# Autodesk Inventor assembly: Frame Assembly - Bade v1
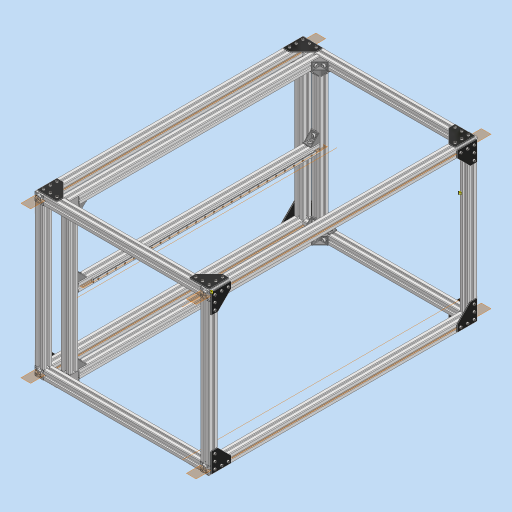
[picture p0: Inventor's stored thumbnail of the model, 512x512]
Saved by Autodesk Inventor 2023.2 (Build 272271000, 271)
## iProperties
Created: 2023-11-22
Part Number: Frame Assembly - Bade v1
Document SubType Name: Assembly
Designer: Nils Bade
Author: Nils Bade
## Documents named in this file (14)
- C:\Users\nilsb\Documents\Inventor\Projektarbeit-Bade\RatRig_Bade\Frame Assembly - Bade v1.iam
- C:\Users\nilsb\Documents\Inventor\Projektarbeit-Bade\RatRig_modified\T-SLOT 4040 B-Type 705mm.ipt
- C:\Users\nilsb\Documents\Inventor\Projektarbeit-Bade\RatRig_modified\T-SLOT 4040 B-Type 640mm.ipt
- C:\Users\nilsb\Documents\Inventor\Projektarbeit-Bade\RatRig_modified\T-SLOT 4040 B-Type 1207mm.ipt
- C:\Users\nilsb\Documents\Inventor\Projektarbeit-Bade\RatRig_modified\T-SLOT 4040 B-Type 1127mm.ipt
- C:\Users\nilsb\Documents\Inventor\Projektarbeit-Bade\RatRig_modified\Joining Plate for 4040 Assembly - A.iam
- C:\Users\nilsb\Documents\Inventor\Projektarbeit-Bade\RatRig_modified\Joining Plate for 4040 Assembly - B.iam
- C:\Users\nilsb\Documents\Inventor\Projektarbeit-Bade\RatRig_modified\Joining Plate for 4040 Assembly - C.iam
- C:\Users\nilsb\Documents\Inventor\Projektarbeit-Bade\RatRig_modified\Joining Plate for 4040 Assembly - A_mir.iam
- C:\Users\nilsb\Documents\Inventor\Projektarbeit-Bade\RatRig_modified\Joining Plate for 4040 Assembly - B_mir.iam
- C:\Users\nilsb\Documents\Inventor\Projektarbeit-Bade\RatRig_modified\Bracket - Cast 90 deg corner 4040 - Assembly.iam
- C:\Users\nilsb\Documents\Inventor\Projektarbeit-Bade\RatRig_modified\T-SLOT 4040 B-Type 1087mm.ipt
- C:\Users\nilsb\Documents\Inventor\Projektarbeit-Bade\RatRig_modified\MGN15 Linear Rail 1000mm - 4040 Assembly.iam
- C:\Users\nilsb\Documents\Inventor\Projektarbeit-Bade\RatRig_modified\MGN15 Linear Rail 550mm - 4040 Assembly.iam
## Components (54 placed, 13 different names)
1. T-SLOT 4040 B-Type 705mm:1 — Passend:1, Passend:2, Passend:3, Passend:6, Passend:7, Passend:8, Fluchtend:6, Fluchtend:8, Fluchtend:9, Fluchtend:14, Passend:14, Fluchtend:19, Fluchtend:20, Passend:15, Passend:20, Fluchtend:29, Passend:51, Passend:53, Passend:54, Passend:62, Passend:63, Passend:115, Passend:117, Passend:119, Fluchtend:39
2. T-SLOT 4040 B-Type 640mm:1 — Passend:6, Fluchtend:8, Passend:17, Fluchtend:22, Fluchtend:23, Passend:40, Passend:41, Passend:55, Passend:56, Passend:57
3. T-SLOT 4040 B-Type 640mm:2 — Passend:7, Fluchtend:9, Passend:9, Fluchtend:26, Fluchtend:27, Passend:108, Passend:110, Passend:111, Passend:113, Passend:114, Passend:116, Passend:123, Passend:125, Passend:139, Passend:140, Passend:141, Passend:142, Fluchtend:40
4. T-SLOT 4040 B-Type 640mm:3 — Passend:8, Fluchtend:6, Passend:9, Fluchtend:16, Passend:16, Fluchtend:21, Fluchtend:24, Passend:31, Passend:32, Passend:48, Passend:52
5. T-SLOT 4040 B-Type 705mm:2 — Fluchtend:14, Passend:18, Passend:19, Fluchtend:25, Passend:21, Fluchtend:28, Passend:49, Passend:50, Passend:58, Passend:59, Passend:70, Passend:71, Passend:74, Passend:75, Passend:120, Passend:122, Passend:124
6. T-SLOT 4040 B-Type 1207mm:1 — Passend:10, Fluchtend:20, Passend:15, Fluchtend:24, Passend:25, Fluchtend:36, Passend:28, Passend:29, Passend:30, Passend:46, Passend:60, Passend:61, Passend:67, Passend:82, Passend:84, Passend:85, Passend:86, Fluchtend:42, Fluchtend:46, Fluchtend:47, Passend:163, Passend:164
7. T-SLOT 4040 B-Type 1207mm:2 — Passend:12, Passend:17, Fluchtend:22, Passend:23, Fluchtend:32, Fluchtend:33, Passend:38, Passend:39, Passend:43, Passend:44, Passend:72, Passend:73, Passend:94, Passend:95, Passend:97, Passend:98
8. T-SLOT 4040 B-Type 1207mm:3 — Passend:13, Passend:16, Fluchtend:21, Passend:19, Fluchtend:25, Fluchtend:34, Passend:33, Passend:34, Passend:35, Passend:47, Passend:68, Passend:69, Passend:89, Passend:90, Passend:91, Passend:92, Fluchtend:43, Fluchtend:44, Fluchtend:48, Passend:162, Passend:165
9. T-SLOT 4040 B-Type 1207mm:4 — Passend:11, Passend:14, Fluchtend:19, Fluchtend:23, Fluchtend:30, Passend:22, Fluchtend:31, Fluchtend:35, Passend:24, Fluchtend:37, Passend:36, Passend:37, Passend:42, Passend:45, Passend:64, Passend:65, Passend:66, Passend:76, Passend:77, Passend:79, Passend:81
10. T-SLOT 4040 B-Type 1127mm:1 — Passend:20, Fluchtend:26, Fluchtend:29, Passend:27, Fluchtend:38, Passend:112, Passend:118, Passend:128, Passend:131
11. T-SLOT 4040 B-Type 1127mm:2 — Passend:21, Fluchtend:27, Fluchtend:28, Passend:109, Passend:121, Passend:134, Passend:137
12. T-SLOT 4040 B-Type 705mm:3 — Fluchtend:30, Passend:22, Fluchtend:31, Passend:26, Passend:80, Passend:83, Passend:103, Passend:104, Passend:126, Passend:127, Passend:150, Passend:155
13. T-SLOT 4040 B-Type 705mm:4 — Passend:23, Fluchtend:32, Fluchtend:33, Passend:93, Passend:96, Passend:100, Passend:107, Passend:132, Passend:133, Passend:151, Passend:154
14. T-SLOT 4040 B-Type 640mm:4 — Fluchtend:35, Passend:24, Fluchtend:37, Passend:78, Passend:99, Passend:101, Passend:102
15. T-SLOT 4040 B-Type 640mm:5 — Fluchtend:34, Passend:25, Fluchtend:36, Passend:87, Passend:88, Passend:105, Passend:106
16. T-SLOT 4040 B-Type 640mm:6 — Passend:26, Passend:27, Fluchtend:38, Passend:129, Passend:130, Passend:135, Passend:136, Passend:144, Passend:146, Fluchtend:41, Fluchtend:45
17. Joining Plate for 4040 Assembly - A:1 [sub-assembly] — Passend:32, Passend:33, Passend:34, Passend:35
18. Joining Plate for 4040 Assembly - B:1 [sub-assembly] — Passend:28, Passend:29, Passend:30, Passend:31
19. Joining Plate for 4040 Assembly - B:3 [sub-assembly] — Passend:38, Passend:39, Passend:40, Passend:43
20. Joining Plate for 4040 Assembly - A:2 [sub-assembly] — Passend:36, Passend:37, Passend:41, Passend:42
21. Joining Plate for 4040 Assembly - C:1 [sub-assembly] — Passend:45, Passend:54, Passend:55, Passend:56
22. Joining Plate for 4040 Assembly - C:2 [sub-assembly] — Passend:44, Passend:57, Passend:58, Passend:59
23. Joining Plate for 4040 Assembly - C:3 [sub-assembly] — Passend:47, Passend:48, Passend:49, Passend:50
24. Joining Plate for 4040 Assembly - C:4 [sub-assembly] — Passend:46, Passend:51, Passend:52, Passend:53
25. Joining Plate for 4040 Assembly - A_mir:1 [sub-assembly] — Passend:63, Passend:64, Passend:65, Passend:66
26. Joining Plate for 4040 Assembly - A_mir:2 [sub-assembly] — Passend:68, Passend:69, Passend:70, Passend:71
27. Joining Plate for 4040 Assembly - B_mir:1 [sub-assembly] — Passend:60, Passend:61, Passend:62, Passend:67
28. Joining Plate for 4040 Assembly - B_mir:2 [sub-assembly] — Passend:72, Passend:73, Passend:74, Passend:75
29. Joining Plate for 4040 Assembly - A:3 [sub-assembly] — Passend:97, Passend:98, Passend:99, Passend:101
30. Joining Plate for 4040 Assembly - B:4 [sub-assembly] — Passend:76, Passend:77, Passend:78, Passend:102
31. Joining Plate for 4040 Assembly - B:5 [sub-assembly] — Passend:88, Passend:89, Passend:90, Passend:106
32. Joining Plate for 4040 Assembly - A:4 [sub-assembly] — Passend:85, Passend:86, Passend:87, Passend:105
33. Joining Plate for 4040 Assembly - A_mir:3 [sub-assembly] — Passend:94, Passend:95, Passend:96, Passend:100
34. Joining Plate for 4040 Assembly - A_mir:4 [sub-assembly] — Passend:82, Passend:83, Passend:84, Passend:104
35. Joining Plate for 4040 Assembly - B_mir:3 [sub-assembly] — Passend:91, Passend:92, Passend:93, Passend:107
36. Joining Plate for 4040 Assembly - B_mir:4 [sub-assembly] — Passend:79, Passend:80, Passend:81, Passend:103
37. Bracket - Cast 90 deg corner 4040 - Assembly:1 [sub-assembly] — Passend:111, Passend:112, Passend:113
38. Bracket - Cast 90 deg corner 4040 - Assembly:2 [sub-assembly] — Passend:108, Passend:109, Passend:110
39. Bracket - Cast 90 deg corner 4040 - Assembly:3 [sub-assembly] — Passend:114, Passend:115, Passend:116
40. Bracket - Cast 90 deg corner 4040 - Assembly:4 [sub-assembly] — Passend:123, Passend:124, Passend:125
41. Bracket - Cast 90 deg corner 4040 - Assembly:5 [sub-assembly] — Passend:120, Passend:121, Passend:122
42. Bracket - Cast 90 deg corner 4040 - Assembly:6 [sub-assembly] — Passend:117, Passend:118, Passend:119
43. Bracket - Cast 90 deg corner 4040 - Assembly:7 [sub-assembly] — Passend:129, Passend:130, Passend:131
44. Bracket - Cast 90 deg corner 4040 - Assembly:8 [sub-assembly] — Passend:135, Passend:136, Passend:137
45. Bracket - Cast 90 deg corner 4040 - Assembly:9 [sub-assembly] — Passend:132, Passend:133, Passend:134, Passend:153
46. Bracket - Cast 90 deg corner 4040 - Assembly:10 [sub-assembly] — Passend:126, Passend:127, Passend:128, Passend:152
47. T-SLOT 4040 B-Type 1087mm:1 — Passend:138, Passend:139, Passend:140, Passend:143, Passend:145, Passend:147, Passend:148
48. Bracket - Cast 90 deg corner 4040 - Assembly:11 [sub-assembly] — Passend:144, Passend:145, Passend:146
49. Bracket - Cast 90 deg corner 4040 - Assembly:12 [sub-assembly] — Passend:141, Passend:142, Passend:143
50. MGN15 Linear Rail 1000mm - 4040 Assembly:1 [sub-assembly] — Passend:147, Passend:148, Passend:149
51. MGN15 Linear Rail 550mm - 4040 Assembly:1 [sub-assembly] — Passend:151, Passend:153, Passend:154
52. MGN15 Linear Rail 550mm - 4040 Assembly:2 [sub-assembly] — Passend:150, Passend:152, Passend:155
53. MGN15 Linear Rail 1000mm - 4040 Assembly:2 [sub-assembly] — Passend:163, Passend:164, Passend:167
54. MGN15 Linear Rail 1000mm - 4040 Assembly:3 [sub-assembly] — Passend:162, Passend:165, Passend:166
## Relationships (202: Mate 165, Flush 37)
- Passend:1 [Mate]: T-SLOT 4040 B-Type 705mm:1
- Passend:2 [Mate]: T-SLOT 4040 B-Type 705mm:1
- Passend:3 [Mate]: T-SLOT 4040 B-Type 705mm:1
- Passend:6 [Mate]: T-SLOT 4040 B-Type 705mm:1 ↔ T-SLOT 4040 B-Type 640mm:1
- Passend:7 [Mate]: T-SLOT 4040 B-Type 705mm:1 ↔ T-SLOT 4040 B-Type 640mm:2
- Passend:8 [Mate]: T-SLOT 4040 B-Type 705mm:1 ↔ T-SLOT 4040 B-Type 640mm:3
- Fluchtend:6 [Flush]: T-SLOT 4040 B-Type 705mm:1 ↔ T-SLOT 4040 B-Type 640mm:3
- Fluchtend:8 [Flush]: T-SLOT 4040 B-Type 705mm:1 ↔ T-SLOT 4040 B-Type 640mm:1
- Fluchtend:9 [Flush]: T-SLOT 4040 B-Type 705mm:1 ↔ T-SLOT 4040 B-Type 640mm:2
- Passend:9 [Mate] (628 mm): T-SLOT 4040 B-Type 640mm:2 ↔ T-SLOT 4040 B-Type 640mm:3
- Fluchtend:14 [Flush]: T-SLOT 4040 B-Type 705mm:1 ↔ T-SLOT 4040 B-Type 705mm:2
- Fluchtend:16 [Flush] (47 mm): T-SLOT 4040 B-Type 640mm:3
- Fluchtend:17 [Flush] (1057 mm)
- Fluchtend:18 [Flush] (63 mm)
- Passend:10 [Mate]: T-SLOT 4040 B-Type 1207mm:1
- Passend:11 [Mate]: T-SLOT 4040 B-Type 1207mm:4
- Passend:12 [Mate]: T-SLOT 4040 B-Type 1207mm:2
- Passend:13 [Mate]: T-SLOT 4040 B-Type 1207mm:3
- Passend:14 [Mate]: T-SLOT 4040 B-Type 705mm:1 ↔ T-SLOT 4040 B-Type 1207mm:4
- Fluchtend:19 [Flush]: T-SLOT 4040 B-Type 705mm:1 ↔ T-SLOT 4040 B-Type 1207mm:4
- Fluchtend:20 [Flush]: T-SLOT 4040 B-Type 705mm:1 ↔ T-SLOT 4040 B-Type 1207mm:1
- Passend:15 [Mate]: T-SLOT 4040 B-Type 705mm:1 ↔ T-SLOT 4040 B-Type 1207mm:1
- Passend:16 [Mate]: T-SLOT 4040 B-Type 640mm:3 ↔ T-SLOT 4040 B-Type 1207mm:3
- Fluchtend:21 [Flush]: T-SLOT 4040 B-Type 640mm:3 ↔ T-SLOT 4040 B-Type 1207mm:3
- Passend:17 [Mate]: T-SLOT 4040 B-Type 640mm:1 ↔ T-SLOT 4040 B-Type 1207mm:2
- Fluchtend:22 [Flush]: T-SLOT 4040 B-Type 640mm:1 ↔ T-SLOT 4040 B-Type 1207mm:2
- Fluchtend:23 [Flush]: T-SLOT 4040 B-Type 640mm:1 ↔ T-SLOT 4040 B-Type 1207mm:4
- Fluchtend:24 [Flush]: T-SLOT 4040 B-Type 640mm:3 ↔ T-SLOT 4040 B-Type 1207mm:1
- Passend:18 [Mate]: T-SLOT 4040 B-Type 705mm:2
- Passend:19 [Mate]: T-SLOT 4040 B-Type 705mm:2 ↔ T-SLOT 4040 B-Type 1207mm:3
- Fluchtend:25 [Flush]: T-SLOT 4040 B-Type 705mm:2 ↔ T-SLOT 4040 B-Type 1207mm:3
- Passend:20 [Mate]: T-SLOT 4040 B-Type 705mm:1 ↔ T-SLOT 4040 B-Type 1127mm:1
- Passend:21 [Mate]: T-SLOT 4040 B-Type 705mm:2 ↔ T-SLOT 4040 B-Type 1127mm:2
- Fluchtend:26 [Flush]: T-SLOT 4040 B-Type 640mm:2 ↔ T-SLOT 4040 B-Type 1127mm:1
- Fluchtend:27 [Flush]: T-SLOT 4040 B-Type 640mm:2 ↔ T-SLOT 4040 B-Type 1127mm:2
- Fluchtend:28 [Flush]: T-SLOT 4040 B-Type 705mm:2 ↔ T-SLOT 4040 B-Type 1127mm:2
- Fluchtend:29 [Flush]: T-SLOT 4040 B-Type 705mm:1 ↔ T-SLOT 4040 B-Type 1127mm:1
- Fluchtend:30 [Flush]: T-SLOT 4040 B-Type 1207mm:4 ↔ T-SLOT 4040 B-Type 705mm:3
- Passend:22 [Mate]: T-SLOT 4040 B-Type 1207mm:4 ↔ T-SLOT 4040 B-Type 705mm:3
- Fluchtend:31 [Flush]: T-SLOT 4040 B-Type 1207mm:4 ↔ T-SLOT 4040 B-Type 705mm:3
- Passend:23 [Mate]: T-SLOT 4040 B-Type 1207mm:2 ↔ T-SLOT 4040 B-Type 705mm:4
- Fluchtend:32 [Flush]: T-SLOT 4040 B-Type 1207mm:2 ↔ T-SLOT 4040 B-Type 705mm:4
- Fluchtend:33 [Flush]: T-SLOT 4040 B-Type 1207mm:2 ↔ T-SLOT 4040 B-Type 705mm:4
- Fluchtend:34 [Flush]: T-SLOT 4040 B-Type 1207mm:3 ↔ T-SLOT 4040 B-Type 640mm:5
- Fluchtend:35 [Flush]: T-SLOT 4040 B-Type 1207mm:4 ↔ T-SLOT 4040 B-Type 640mm:4
- Passend:24 [Mate]: T-SLOT 4040 B-Type 1207mm:4 ↔ T-SLOT 4040 B-Type 640mm:4
- Passend:25 [Mate]: T-SLOT 4040 B-Type 1207mm:1 ↔ T-SLOT 4040 B-Type 640mm:5
- Fluchtend:36 [Flush]: T-SLOT 4040 B-Type 1207mm:1 ↔ T-SLOT 4040 B-Type 640mm:5
- Fluchtend:37 [Flush]: T-SLOT 4040 B-Type 1207mm:4 ↔ T-SLOT 4040 B-Type 640mm:4
- Passend:26 [Mate]: T-SLOT 4040 B-Type 705mm:3 ↔ T-SLOT 4040 B-Type 640mm:6
- Passend:27 [Mate]: T-SLOT 4040 B-Type 1127mm:1 ↔ T-SLOT 4040 B-Type 640mm:6
- Fluchtend:38 [Flush]: T-SLOT 4040 B-Type 1127mm:1 ↔ T-SLOT 4040 B-Type 640mm:6
- Passend:28 [Mate]: T-SLOT 4040 B-Type 1207mm:1 ↔ Joining Plate for 4040 Assembly - B:1
- Passend:29 [Mate]: T-SLOT 4040 B-Type 1207mm:1 ↔ Joining Plate for 4040 Assembly - B:1
- Passend:30 [Mate]: T-SLOT 4040 B-Type 1207mm:1 ↔ Joining Plate for 4040 Assembly - B:1
- Passend:31 [Mate]: T-SLOT 4040 B-Type 640mm:3 ↔ Joining Plate for 4040 Assembly - B:1
- Passend:32 [Mate]: T-SLOT 4040 B-Type 640mm:3 ↔ Joining Plate for 4040 Assembly - A:1
- Passend:33 [Mate]: T-SLOT 4040 B-Type 1207mm:3 ↔ Joining Plate for 4040 Assembly - A:1
- Passend:34 [Mate]: T-SLOT 4040 B-Type 1207mm:3 ↔ Joining Plate for 4040 Assembly - A:1
- Passend:35 [Mate]: T-SLOT 4040 B-Type 1207mm:3 ↔ Joining Plate for 4040 Assembly - A:1
- Passend:36 [Mate]: T-SLOT 4040 B-Type 1207mm:4 ↔ Joining Plate for 4040 Assembly - A:2
- Passend:37 [Mate]: T-SLOT 4040 B-Type 1207mm:4 ↔ Joining Plate for 4040 Assembly - A:2
- Passend:38 [Mate]: T-SLOT 4040 B-Type 1207mm:2 ↔ Joining Plate for 4040 Assembly - B:3
- Passend:39 [Mate]: T-SLOT 4040 B-Type 1207mm:2 ↔ Joining Plate for 4040 Assembly - B:3
- Passend:40 [Mate]: T-SLOT 4040 B-Type 640mm:1 ↔ Joining Plate for 4040 Assembly - B:3
- Passend:41 [Mate]: T-SLOT 4040 B-Type 640mm:1 ↔ Joining Plate for 4040 Assembly - A:2
- Passend:42 [Mate]: T-SLOT 4040 B-Type 1207mm:4 ↔ Joining Plate for 4040 Assembly - A:2
- Passend:43 [Mate]: T-SLOT 4040 B-Type 1207mm:2 ↔ Joining Plate for 4040 Assembly - B:3
- Passend:44 [Mate]: T-SLOT 4040 B-Type 1207mm:2 ↔ Joining Plate for 4040 Assembly - C:2
- Passend:45 [Mate]: T-SLOT 4040 B-Type 1207mm:4 ↔ Joining Plate for 4040 Assembly - C:1
- Passend:46 [Mate]: T-SLOT 4040 B-Type 1207mm:1 ↔ Joining Plate for 4040 Assembly - C:4
- Passend:47 [Mate]: T-SLOT 4040 B-Type 1207mm:3 ↔ Joining Plate for 4040 Assembly - C:3
- Passend:48 [Mate]: T-SLOT 4040 B-Type 640mm:3 ↔ Joining Plate for 4040 Assembly - C:3
- Passend:49 [Mate]: T-SLOT 4040 B-Type 705mm:2 ↔ Joining Plate for 4040 Assembly - C:3
- Passend:50 [Mate]: T-SLOT 4040 B-Type 705mm:2 ↔ Joining Plate for 4040 Assembly - C:3
- Passend:51 [Mate]: T-SLOT 4040 B-Type 705mm:1 ↔ Joining Plate for 4040 Assembly - C:4
- Passend:52 [Mate]: T-SLOT 4040 B-Type 640mm:3 ↔ Joining Plate for 4040 Assembly - C:4
- Passend:53 [Mate]: T-SLOT 4040 B-Type 705mm:1 ↔ Joining Plate for 4040 Assembly - C:4
- Passend:54 [Mate]: T-SLOT 4040 B-Type 705mm:1 ↔ Joining Plate for 4040 Assembly - C:1
- Passend:55 [Mate]: T-SLOT 4040 B-Type 640mm:1 ↔ Joining Plate for 4040 Assembly - C:1
- Passend:56 [Mate]: T-SLOT 4040 B-Type 640mm:1 ↔ Joining Plate for 4040 Assembly - C:1
- Passend:57 [Mate]: T-SLOT 4040 B-Type 640mm:1 ↔ Joining Plate for 4040 Assembly - C:2
- Passend:58 [Mate]: T-SLOT 4040 B-Type 705mm:2 ↔ Joining Plate for 4040 Assembly - C:2
- Passend:59 [Mate]: T-SLOT 4040 B-Type 705mm:2 ↔ Joining Plate for 4040 Assembly - C:2
- Passend:60 [Mate]: T-SLOT 4040 B-Type 1207mm:1 ↔ Joining Plate for 4040 Assembly - B_mir:1
- Passend:61 [Mate]: T-SLOT 4040 B-Type 1207mm:1 ↔ Joining Plate for 4040 Assembly - B_mir:1
- Passend:62 [Mate]: T-SLOT 4040 B-Type 705mm:1 ↔ Joining Plate for 4040 Assembly - B_mir:1
- Passend:63 [Mate]: T-SLOT 4040 B-Type 705mm:1 ↔ Joining Plate for 4040 Assembly - A_mir:1
- Passend:64 [Mate]: T-SLOT 4040 B-Type 1207mm:4 ↔ Joining Plate for 4040 Assembly - A_mir:1
- Passend:65 [Mate]: T-SLOT 4040 B-Type 1207mm:4 ↔ Joining Plate for 4040 Assembly - A_mir:1
- Passend:66 [Mate]: T-SLOT 4040 B-Type 1207mm:4 ↔ Joining Plate for 4040 Assembly - A_mir:1
- Passend:67 [Mate]: T-SLOT 4040 B-Type 1207mm:1 ↔ Joining Plate for 4040 Assembly - B_mir:1
- Passend:68 [Mate]: T-SLOT 4040 B-Type 1207mm:3 ↔ Joining Plate for 4040 Assembly - A_mir:2
- Passend:69 [Mate]: T-SLOT 4040 B-Type 1207mm:3 ↔ Joining Plate for 4040 Assembly - A_mir:2
- Passend:70 [Mate]: T-SLOT 4040 B-Type 705mm:2 ↔ Joining Plate for 4040 Assembly - A_mir:2
- Passend:71 [Mate]: T-SLOT 4040 B-Type 705mm:2 ↔ Joining Plate for 4040 Assembly - A_mir:2
- Passend:72 [Mate]: T-SLOT 4040 B-Type 1207mm:2 ↔ Joining Plate for 4040 Assembly - B_mir:2
- Passend:73 [Mate]: T-SLOT 4040 B-Type 1207mm:2 ↔ Joining Plate for 4040 Assembly - B_mir:2
- Passend:74 [Mate]: T-SLOT 4040 B-Type 705mm:2 ↔ Joining Plate for 4040 Assembly - B_mir:2
- Passend:75 [Mate]: T-SLOT 4040 B-Type 705mm:2 ↔ Joining Plate for 4040 Assembly - B_mir:2
- Passend:76 [Mate]: T-SLOT 4040 B-Type 1207mm:4 ↔ Joining Plate for 4040 Assembly - B:4
- Passend:77 [Mate]: T-SLOT 4040 B-Type 1207mm:4 ↔ Joining Plate for 4040 Assembly - B:4
- Passend:78 [Mate]: T-SLOT 4040 B-Type 640mm:4 ↔ Joining Plate for 4040 Assembly - B:4
- Passend:79 [Mate]: T-SLOT 4040 B-Type 1207mm:4 ↔ Joining Plate for 4040 Assembly - B_mir:4
- Passend:80 [Mate]: T-SLOT 4040 B-Type 705mm:3 ↔ Joining Plate for 4040 Assembly - B_mir:4
- Passend:81 [Mate]: T-SLOT 4040 B-Type 1207mm:4 ↔ Joining Plate for 4040 Assembly - B_mir:4
- Passend:82 [Mate]: T-SLOT 4040 B-Type 1207mm:1 ↔ Joining Plate for 4040 Assembly - A_mir:4
- Passend:83 [Mate]: T-SLOT 4040 B-Type 705mm:3 ↔ Joining Plate for 4040 Assembly - A_mir:4
- Passend:84 [Mate]: T-SLOT 4040 B-Type 1207mm:1 ↔ Joining Plate for 4040 Assembly - A_mir:4
- Passend:85 [Mate]: T-SLOT 4040 B-Type 1207mm:1 ↔ Joining Plate for 4040 Assembly - A:4
- Passend:86 [Mate]: T-SLOT 4040 B-Type 1207mm:1 ↔ Joining Plate for 4040 Assembly - A:4
- Passend:87 [Mate]: T-SLOT 4040 B-Type 640mm:5 ↔ Joining Plate for 4040 Assembly - A:4
- Passend:88 [Mate]: T-SLOT 4040 B-Type 640mm:5 ↔ Joining Plate for 4040 Assembly - B:5
- Passend:89 [Mate]: T-SLOT 4040 B-Type 1207mm:3 ↔ Joining Plate for 4040 Assembly - B:5
- Passend:90 [Mate]: T-SLOT 4040 B-Type 1207mm:3 ↔ Joining Plate for 4040 Assembly - B:5
- Passend:91 [Mate]: T-SLOT 4040 B-Type 1207mm:3 ↔ Joining Plate for 4040 Assembly - B_mir:3
- Passend:92 [Mate]: T-SLOT 4040 B-Type 1207mm:3 ↔ Joining Plate for 4040 Assembly - B_mir:3
- Passend:93 [Mate]: T-SLOT 4040 B-Type 705mm:4 ↔ Joining Plate for 4040 Assembly - B_mir:3
- Passend:94 [Mate]: T-SLOT 4040 B-Type 1207mm:2 ↔ Joining Plate for 4040 Assembly - A_mir:3
- Passend:95 [Mate]: T-SLOT 4040 B-Type 1207mm:2 ↔ Joining Plate for 4040 Assembly - A_mir:3
- Passend:96 [Mate]: T-SLOT 4040 B-Type 705mm:4 ↔ Joining Plate for 4040 Assembly - A_mir:3
- Passend:97 [Mate]: T-SLOT 4040 B-Type 1207mm:2 ↔ Joining Plate for 4040 Assembly - A:3
- Passend:98 [Mate]: T-SLOT 4040 B-Type 1207mm:2 ↔ Joining Plate for 4040 Assembly - A:3
- Passend:99 [Mate]: T-SLOT 4040 B-Type 640mm:4 ↔ Joining Plate for 4040 Assembly - A:3
- Passend:100 [Mate]: T-SLOT 4040 B-Type 705mm:4 ↔ Joining Plate for 4040 Assembly - A_mir:3
- Passend:101 [Mate]: T-SLOT 4040 B-Type 640mm:4 ↔ Joining Plate for 4040 Assembly - A:3
- Passend:102 [Mate]: T-SLOT 4040 B-Type 640mm:4 ↔ Joining Plate for 4040 Assembly - B:4
- Passend:103 [Mate]: T-SLOT 4040 B-Type 705mm:3 ↔ Joining Plate for 4040 Assembly - B_mir:4
- Passend:104 [Mate]: T-SLOT 4040 B-Type 705mm:3 ↔ Joining Plate for 4040 Assembly - A_mir:4
- Passend:105 [Mate]: T-SLOT 4040 B-Type 640mm:5 ↔ Joining Plate for 4040 Assembly - A:4
- Passend:106 [Mate]: T-SLOT 4040 B-Type 640mm:5 ↔ Joining Plate for 4040 Assembly - B:5
- Passend:107 [Mate]: T-SLOT 4040 B-Type 705mm:4 ↔ Joining Plate for 4040 Assembly - B_mir:3
- Passend:108 [Mate]: T-SLOT 4040 B-Type 640mm:2 ↔ Bracket - Cast 90 deg corner 4040 - Assembly:2
- Passend:109 [Mate]: T-SLOT 4040 B-Type 1127mm:2 ↔ Bracket - Cast 90 deg corner 4040 - Assembly:2
- Passend:110 [Mate]: T-SLOT 4040 B-Type 640mm:2 ↔ Bracket - Cast 90 deg corner 4040 - Assembly:2
- Passend:111 [Mate]: T-SLOT 4040 B-Type 640mm:2 ↔ Bracket - Cast 90 deg corner 4040 - Assembly:1
- Passend:112 [Mate]: T-SLOT 4040 B-Type 1127mm:1 ↔ Bracket - Cast 90 deg corner 4040 - Assembly:1
- Passend:113 [Mate]: T-SLOT 4040 B-Type 640mm:2 ↔ Bracket - Cast 90 deg corner 4040 - Assembly:1
- Passend:114 [Mate]: T-SLOT 4040 B-Type 640mm:2 ↔ Bracket - Cast 90 deg corner 4040 - Assembly:3
- Passend:115 [Mate]: T-SLOT 4040 B-Type 705mm:1 ↔ Bracket - Cast 90 deg corner 4040 - Assembly:3
- Passend:116 [Mate]: T-SLOT 4040 B-Type 640mm:2 ↔ Bracket - Cast 90 deg corner 4040 - Assembly:3
- Passend:117 [Mate]: T-SLOT 4040 B-Type 705mm:1 ↔ Bracket - Cast 90 deg corner 4040 - Assembly:6
- Passend:118 [Mate]: T-SLOT 4040 B-Type 1127mm:1 ↔ Bracket - Cast 90 deg corner 4040 - Assembly:6
- Passend:119 [Mate]: T-SLOT 4040 B-Type 705mm:1 ↔ Bracket - Cast 90 deg corner 4040 - Assembly:6
- Passend:120 [Mate]: T-SLOT 4040 B-Type 705mm:2 ↔ Bracket - Cast 90 deg corner 4040 - Assembly:5
- Passend:121 [Mate]: T-SLOT 4040 B-Type 1127mm:2 ↔ Bracket - Cast 90 deg corner 4040 - Assembly:5
- Passend:122 [Mate]: T-SLOT 4040 B-Type 705mm:2 ↔ Bracket - Cast 90 deg corner 4040 - Assembly:5
- Passend:123 [Mate]: T-SLOT 4040 B-Type 640mm:2 ↔ Bracket - Cast 90 deg corner 4040 - Assembly:4
- Passend:124 [Mate]: T-SLOT 4040 B-Type 705mm:2 ↔ Bracket - Cast 90 deg corner 4040 - Assembly:4
- Passend:125 [Mate]: T-SLOT 4040 B-Type 640mm:2 ↔ Bracket - Cast 90 deg corner 4040 - Assembly:4
- Passend:126 [Mate]: T-SLOT 4040 B-Type 705mm:3 ↔ Bracket - Cast 90 deg corner 4040 - Assembly:10
- Passend:127 [Mate]: T-SLOT 4040 B-Type 705mm:3 ↔ Bracket - Cast 90 deg corner 4040 - Assembly:10
- Passend:128 [Mate]: T-SLOT 4040 B-Type 1127mm:1 ↔ Bracket - Cast 90 deg corner 4040 - Assembly:10
- Passend:129 [Mate]: T-SLOT 4040 B-Type 640mm:6 ↔ Bracket - Cast 90 deg corner 4040 - Assembly:7
- Passend:130 [Mate]: T-SLOT 4040 B-Type 640mm:6 ↔ Bracket - Cast 90 deg corner 4040 - Assembly:7
- Passend:131 [Mate]: T-SLOT 4040 B-Type 1127mm:1 ↔ Bracket - Cast 90 deg corner 4040 - Assembly:7
- Passend:132 [Mate]: T-SLOT 4040 B-Type 705mm:4 ↔ Bracket - Cast 90 deg corner 4040 - Assembly:9
- Passend:133 [Mate]: T-SLOT 4040 B-Type 705mm:4 ↔ Bracket - Cast 90 deg corner 4040 - Assembly:9
- Passend:134 [Mate]: T-SLOT 4040 B-Type 1127mm:2 ↔ Bracket - Cast 90 deg corner 4040 - Assembly:9
- Passend:135 [Mate]: T-SLOT 4040 B-Type 640mm:6 ↔ Bracket - Cast 90 deg corner 4040 - Assembly:8
- Passend:136 [Mate]: T-SLOT 4040 B-Type 640mm:6 ↔ Bracket - Cast 90 deg corner 4040 - Assembly:8
- Passend:137 [Mate]: T-SLOT 4040 B-Type 1127mm:2 ↔ Bracket - Cast 90 deg corner 4040 - Assembly:8
- Fluchtend:39 [Flush] (320 mm): T-SLOT 4040 B-Type 705mm:1
- Passend:138 [Mate]: T-SLOT 4040 B-Type 1087mm:1
- Passend:139 [Mate]: T-SLOT 4040 B-Type 640mm:2 ↔ T-SLOT 4040 B-Type 1087mm:1
- Passend:140 [Mate]: T-SLOT 4040 B-Type 640mm:2 ↔ T-SLOT 4040 B-Type 1087mm:1
- Passend:141 [Mate]: T-SLOT 4040 B-Type 640mm:2 ↔ Bracket - Cast 90 deg corner 4040 - Assembly:12
- Passend:142 [Mate]: T-SLOT 4040 B-Type 640mm:2 ↔ Bracket - Cast 90 deg corner 4040 - Assembly:12
- Passend:143 [Mate]: T-SLOT 4040 B-Type 1087mm:1 ↔ Bracket - Cast 90 deg corner 4040 - Assembly:12
- Passend:144 [Mate]: T-SLOT 4040 B-Type 640mm:6 ↔ Bracket - Cast 90 deg corner 4040 - Assembly:11
- Passend:145 [Mate]: T-SLOT 4040 B-Type 1087mm:1 ↔ Bracket - Cast 90 deg corner 4040 - Assembly:11
- Passend:146 [Mate]: T-SLOT 4040 B-Type 640mm:6 ↔ Bracket - Cast 90 deg corner 4040 - Assembly:11
- Fluchtend:40 [Flush] (27 mm): T-SLOT 4040 B-Type 640mm:2
- Passend:147 [Mate]: T-SLOT 4040 B-Type 1087mm:1 ↔ MGN15 Linear Rail 1000mm - 4040 Assembly:1
- Passend:148 [Mate]: T-SLOT 4040 B-Type 1087mm:1 ↔ MGN15 Linear Rail 1000mm - 4040 Assembly:1
- Passend:149 [Mate]: MGN15 Linear Rail 1000mm - 4040 Assembly:1
- Passend:150 [Mate]: T-SLOT 4040 B-Type 705mm:3 ↔ MGN15 Linear Rail 550mm - 4040 Assembly:2
- Passend:151 [Mate]: T-SLOT 4040 B-Type 705mm:4 ↔ MGN15 Linear Rail 550mm - 4040 Assembly:1
- Passend:152 [Mate]: Bracket - Cast 90 deg corner 4040 - Assembly:10 ↔ MGN15 Linear Rail 550mm - 4040 Assembly:2
- Passend:153 [Mate]: Bracket - Cast 90 deg corner 4040 - Assembly:9 ↔ MGN15 Linear Rail 550mm - 4040 Assembly:1
- Passend:154 [Mate]: T-SLOT 4040 B-Type 705mm:4 ↔ MGN15 Linear Rail 550mm - 4040 Assembly:1
- Passend:155 [Mate]: T-SLOT 4040 B-Type 705mm:3 ↔ MGN15 Linear Rail 550mm - 4040 Assembly:2
- Fluchtend:41 [Flush] (70 mm): T-SLOT 4040 B-Type 640mm:6
- Fluchtend:42 [Flush] (51.86 mm): T-SLOT 4040 B-Type 1207mm:1
- Fluchtend:43 [Flush] (51.86 mm): T-SLOT 4040 B-Type 1207mm:3
- Fluchtend:44 [Flush] (25.242 mm): T-SLOT 4040 B-Type 1207mm:3
- Fluchtend:45 [Flush] (35.5 mm): T-SLOT 4040 B-Type 640mm:6
- Passend:156 [Mate]
- Passend:157 [Mate]
- Fluchtend:46 [Flush] (21.5 mm): T-SLOT 4040 B-Type 1207mm:1
- Fluchtend:47 [Flush] (21.5 mm): T-SLOT 4040 B-Type 1207mm:1
- Fluchtend:48 [Flush] (21.5 mm): T-SLOT 4040 B-Type 1207mm:3
- Passend:158 [Mate]
- Passend:159 [Mate]
- Passend:160 [Mate]
- Passend:161 [Mate]
- Passend:162 [Mate]: T-SLOT 4040 B-Type 1207mm:3 ↔ MGN15 Linear Rail 1000mm - 4040 Assembly:3
- Passend:163 [Mate]: T-SLOT 4040 B-Type 1207mm:1 ↔ MGN15 Linear Rail 1000mm - 4040 Assembly:2
- Passend:164 [Mate]: T-SLOT 4040 B-Type 1207mm:1 ↔ MGN15 Linear Rail 1000mm - 4040 Assembly:2
- Passend:165 [Mate]: T-SLOT 4040 B-Type 1207mm:3 ↔ MGN15 Linear Rail 1000mm - 4040 Assembly:3
- Passend:166 [Mate]: MGN15 Linear Rail 1000mm - 4040 Assembly:3
- Passend:167 [Mate]: MGN15 Linear Rail 1000mm - 4040 Assembly:2
